# Autodesk Inventor assembly: FumeBOT
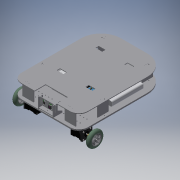
[picture p0: Inventor's stored thumbnail of the model, 180x180]
Saved by Autodesk Inventor 2018 (Build 220112000, 112)
## iProperties
Created: 2018-05-02
Part Number: FumeBOT
Document SubType Name: Assembly
Designer: Ajith Thomas
Author: Ajith Thomas
## Documents named in this file (13)
- C:\Users\Ajith Thomas\Dropbox\Gas_Sensing_Robot\FumeBot-Design\FumeBOT.iam
- C:\Users\Ajith Thomas\Dropbox\Gas_Sensing_Robot\FumeBot-Design\Base.ipt
- C:\Users\Ajith Thomas\Dropbox\Gas_Sensing_Robot\FumeBot-Design\Sensors and Boards\Raspberry Pi 3B.ipt
- C:\Users\Ajith Thomas\Dropbox\Gas_Sensing_Robot\FumeBot-Design\Sensors and Boards\Arduino MEGA 2560 R3\Arduino MEGA 2560 R3.iam
- C:\Users\Ajith Thomas\Dropbox\Gas_Sensing_Robot\FumeBot-Design\Large Bread Board.ipt
- C:\Users\Ajith Thomas\Dropbox\Gas_Sensing_Robot\FumeBot-Design\Small Bread Board.ipt
- C:\Users\Ajith Thomas\Dropbox\Gas_Sensing_Robot\FumeBot-Design\Battery.ipt
- C:\Users\Ajith Thomas\Dropbox\Gas_Sensing_Robot\FumeBot-Design\Stepper with bracket.iam
- C:\Users\Ajith Thomas\Dropbox\Gas_Sensing_Robot\FumeBot-Design\Wheel height spacers.ipt
- C:\Users\Ajith Thomas\Dropbox\Gas_Sensing_Robot\FumeBot-Design\Mecanum with supports.iam
- C:\Users\Ajith Thomas\Dropbox\Gas_Sensing_Robot\FumeBot-Design\Camera mount assembly.iam
- C:\Users\Ajith Thomas\Dropbox\Gas_Sensing_Robot\FumeBot-Design\Base and top seperator.ipt
- C:\Users\Ajith Thomas\Dropbox\Gas_Sensing_Robot\FumeBot-Design\Top plate.ipt
## Components (19 placed, 12 different names)
1. Base:1 — Mate:1, Mate:2, Flush:1, Flush:2, Flush:3, Flush:4, Mate:4, Mate:5, Mate:6, Flush:6, Flush:7, Mate:7, Mate:8, Mate:9, Mate:10, Mate:11, Mate:12, Flush:8, Flush:9, Flush:10, Flush:11, Flush:12, Flush:13, Flush:14, Flush:15, Flush:16, Flush:17, Flush:18, Flush:19, Mate:13, Mate:14, Flush:20, Mate:15, Mate:16, Flush:21, Mate:17, Mate:18
2. Raspberry Pi 3B:1 — Mate:10
3. Arduino MEGA 2560 R3:1 [sub-assembly] — Mate:9
4. Large Bread Board:1 — Mate:8
5. Small Bread Board:1 — Mate:11
6. Battery:1 — Mate:7
7. Stepper with bracket:1 [sub-assembly] — Mate:1, Flush:1, Flush:3, Flush:5
8. Stepper with bracket:2 [sub-assembly] — Mate:2, Flush:2, Flush:4, Mate:3
9. Wheel height spacers:1 — Flush:5
10. Wheel height spacers:2 — Mate:3, Mate:4, Mate:5
11. Mecanum with supports:1 [sub-assembly] — Mate:6, Flush:6, Flush:7
12. Camera mount assembly:1 [sub-assembly] — Mate:12, Flush:8, Flush:9
13. Base and top seperator:1 — Flush:10, Flush:12, Flush:13
14. Base and top seperator:2 — Flush:11, Flush:14, Flush:15
15. Base and top seperator:3 — Flush:16, Flush:17, Flush:18
16. Base and top seperator:4 — Flush:19, Mate:13, Mate:14
17. Base and top seperator:5 — Flush:20, Mate:15, Mate:16, Flush:22
18. Base and top seperator:6 — Flush:21, Mate:17, Mate:18
19. Top plate:1 — Flush:22
## Relationships (40: Flush 22, Mate 18)
- Mate:1 (6 mm): Base:1 ↔ Stepper with bracket:1
- Mate:2 (6 mm): Base:1 ↔ Stepper with bracket:2
- Flush:1 (20 mm): Base:1 ↔ Stepper with bracket:1
- Flush:2 (20 mm): Base:1 ↔ Stepper with bracket:2
- Flush:3 (30 mm): Base:1 ↔ Stepper with bracket:1
- Flush:4 (30 mm): Base:1 ↔ Stepper with bracket:2
- Flush:5: Stepper with bracket:1 ↔ Wheel height spacers:1
- Mate:3: Stepper with bracket:2 ↔ Wheel height spacers:2
- Mate:4: Base:1 ↔ Wheel height spacers:2
- Mate:5: Base:1 ↔ Wheel height spacers:2
- Mate:6: Base:1 ↔ Mecanum with supports:1
- Flush:6 (23 mm): Base:1 ↔ Mecanum with supports:1
- Flush:7 (121.1 mm): Base:1 ↔ Mecanum with supports:1
- Mate:7: Base:1 ↔ Battery:1
- Mate:8: Base:1 ↔ Large Bread Board:1
- Mate:9: Base:1 ↔ Arduino MEGA 2560 R3:1
- Mate:10: Base:1 ↔ Raspberry Pi 3B:1
- Mate:11: Base:1 ↔ Small Bread Board:1
- Mate:12: Base:1 ↔ Camera mount assembly:1
- Flush:8: Base:1 ↔ Camera mount assembly:1
- Flush:9 (115.25 mm): Base:1 ↔ Camera mount assembly:1
- Flush:10: Base:1 ↔ Base and top seperator:1
- Flush:11: Base:1 ↔ Base and top seperator:2
- Flush:12 (15 mm): Base:1 ↔ Base and top seperator:1
- Flush:13 (100 mm): Base:1 ↔ Base and top seperator:1
- Flush:14 (15 mm): Base:1 ↔ Base and top seperator:2
- Flush:15 (50 mm): Base:1 ↔ Base and top seperator:2
- Flush:16: Base:1 ↔ Base and top seperator:3
- Flush:17 (15 mm): Base:1 ↔ Base and top seperator:3
- Flush:18 (30 mm): Base:1 ↔ Base and top seperator:3
- Flush:19: Base:1 ↔ Base and top seperator:4
- Mate:13: Base:1 ↔ Base and top seperator:4
- Mate:14: Base:1 ↔ Base and top seperator:4
- Flush:20: Base:1 ↔ Base and top seperator:5
- Mate:15: Base:1 ↔ Base and top seperator:5
- Mate:16: Base:1 ↔ Base and top seperator:5
- Flush:21: Base:1 ↔ Base and top seperator:6
- Mate:17: Base:1 ↔ Base and top seperator:6
- Mate:18: Base:1 ↔ Base and top seperator:6
- Flush:22: Base and top seperator:5 ↔ Top plate:1
